# Autodesk Inventor assembly: 실리콘틀
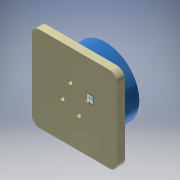
[picture p0: Inventor's stored thumbnail of the model, 180x180]
Saved by Autodesk Inventor 2017 (Build 210142000, 142)
## iProperties
Part Number: 실리콘틀
Material: 일반
Document SubType Name: Assembly
Designer: minom
Author: minom
## Documents named in this file (3)
- C:\Users\minom\Documents\Inventor\Projects\2017 IRC Sumo Mino ver.2\실리콘틀.iam
- C:\Users\minom\Documents\Inventor\Projects\2017 IRC Sumo Mino ver.2\실리콘틀_위.ipt
- C:\Users\minom\Documents\Inventor\Projects\2017 IRC Sumo Mino ver.2\실리콘틀_밑판.ipt
## Components (2 placed, 2 different names)
1. 실리콘틀_위:1 — 메이트:4
2. 실리콘틀_밑판:1 — 메이트:1, 메이트:2, 메이트:3, 메이트:4
## Relationships (4: Mate 4)
- 메이트:1 [Mate]: 실리콘틀_밑판:1
- 메이트:2 [Mate]: 실리콘틀_밑판:1
- 메이트:3 [Mate]: 실리콘틀_밑판:1
- 메이트:4 [Mate]: 실리콘틀_위:1 ↔ 실리콘틀_밑판:1
